# Autodesk Inventor assembly: Papa Cerdito
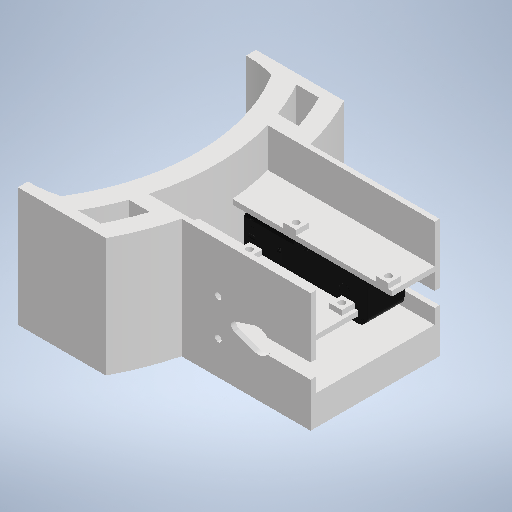
[picture p0: Inventor's stored thumbnail of the model, 512x512]
Saved by Autodesk Inventor 2025.2 (Build 292293000, 293)
## iProperties
Created: 2025-04-24
Part Number: Papa Cerdito
Document SubType Name: Assembly
Designer: thmrc
Author: thmrc
## Documents named in this file (4)
- C:\misa\mecatronics\NOVA\Papa Cerdito - Soccer\Papa Cerdito - Design Mechanical\Papa Cerdito.iam
- C:\misa\mecatronics\NOVA\Papa Cerdito - Soccer\Papa Cerdito - Design Mechanical\Chasis.ipt
- C:\misa\mecatronics\NOVA\Papa Cerdito - Soccer\Papa Cerdito - Design Mechanical\Components\Motor.ipt
- C:\misa\mecatronics\NOVA\Papa Cerdito - Soccer\Papa Cerdito - Design Mechanical\Components\Wheel.ipt
## Components (3 placed, 3 different names)
1. Chasis:1 — Coincidencia:1, Coincidencia:2, Coincidencia:3, Coincidencia:7, Coincidencia:8, Coincidencia:9
2. Motor:1 — Coincidencia:5, Coincidencia:6, Coincidencia:7, Coincidencia:8, Coincidencia:9
3. Wheel:1 — Coincidencia:5, Coincidencia:6
## Relationships (8: Mate 8)
- Coincidencia:1 [Mate]: Chasis:1
- Coincidencia:2 [Mate]: Chasis:1
- Coincidencia:3 [Mate]: Chasis:1
- Coincidencia:5 [Mate]: Motor:1 ↔ Wheel:1
- Coincidencia:6 [Mate] (4 mm): Motor:1 ↔ Wheel:1
- Coincidencia:7 [Mate]: Chasis:1 ↔ Motor:1
- Coincidencia:8 [Mate]: Chasis:1 ↔ Motor:1
- Coincidencia:9 [Mate] (15 mm): Chasis:1 ↔ Motor:1
